# Autodesk Inventor assembly: 51200
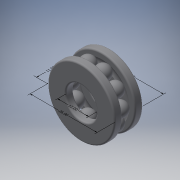
[picture p0: Inventor's stored thumbnail of the model, 180x180]
Saved by Autodesk Inventor 2019 (Build 230136000, 136)
## iProperties
Category: PARTsolutions
Company: NSK_RB
Created: 2023-01-10
Part Number: 51200
Catalog Web Link: www.cadenas.de
Description: With Flat Seet-
Vendor: NSK_RB
Document SubType Name: Assembly
Designer: psAdmin
Manufacturer: NSK_RB
Mass: 28 g
Surface Area: 32.9305 cm^2
Volume: 3.43224 cm^3
Density: 8.15795 g/cm^3
Title: 51200
Author: Cadenas PARTsolutions
PSOL_IDENT_0: {$CADENAS_DATA/23d-libs/nsk_rb/roller_bearings/thrust_bearings/single_direction_tbb/with_flat_seet_a
PSOL_IDENT_1: smtab.prj},174 {VTYP=3D},{STYP=ASSTAB},{NB=51200},{LINA=51200},{NN=With Flat Seet},{DATE=27.09.2022
PSOL_IDENT_2: 23:23:10},{GEOMDATE=23.08.2022 10:47:17},{VERSION=},{LINEID=6260},{WBVAR=},{WBNUMERIC=}  {NB=51200},
PSOL_IDENT_3: {LINA=51200},{KT=DUMMY},{IDNR=},{STAN=Standard},{NO=2},{ORDER=51200},{SD=10},{D=26},{T=11},{T3=11.6}
PSOL_IDENT_4: ,{T4=13},{SR=0.6},{CAN=12800},{COAN=17100},{CA=1300},{COA=1740},{GRE=6000},{OIL=9000},{SD1=26},{D1=1
PSOL_IDENT_5: 2},{D2=18},{D3=28},{SB=3.5},{A=8.5},{R=22},{SDA=20},{DA=16},{SRA=0.6},{MASS=0.028},{PPATH=with_flat_
PSOL_IDENT_6: seet_asmtpl.prj},{N=10},{DIST=1.233}
NB: 51200
NN: With Flat Seet
NBSYN: $ORDER.
LINA: 51200
CATALOG: NSK Rolling Bearing
ORDER: 51200
SD: 10
D: 26
T: 11
SR: 0.6
CAN: 12800
COAN: 17100
CA: 1300
COA: 1740
GRE: 6000
OIL: 9000
SD1: 26
D1: 12
SDA: 20
DA: 16
SRA: 0.6
MASS: 0.028
SUPPLIER: NSK_RB
ARTICLENO: 51200
BOMINFO: 51200
CREATOR: CADENAS GmbH
## Documents named in this file (4)
- e:\temp\worker_COMMON_5\temp\tmp_3544_152_Vz12m\format_0\51200.iam
- e:\temp\worker_COMMON_5\temp\tmp_3544_152_Vz12m\format_0\51200 Housing washer.ipt
- e:\temp\worker_COMMON_5\temp\tmp_3544_152_Vz12m\format_0\51200 Shaft washer.ipt
- e:\temp\worker_COMMON_5\temp\tmp_3544_152_Vz12m\format_0\51200 Ball.ipt
## Components (12 placed, 3 different names)
1. 51200 Housing washer:1 — HW_SW_XY@1 <-> SW_HW_XY@2, HW_SW_Z@1 <-> SW_HW_Z@2, HW_B_1_XY@1 <-> B_HW_XY@3, HW_B_1_Z@1 <-> B_HW_Z@3, HW_B_1_YZ@1 <-> B_HW_YZ@3, HW_B_2_XY@1 <-> B_HW_XY@4, HW_B_2_Z@1 <-> B_HW_Z@4, HW_B_2_YZ@1 <-> B_HW_YZ@4, HW_B_3_XY@1 <-> B_HW_XY@5, HW_B_3_Z@1 <-> B_HW_Z@5, HW_B_3_YZ@1 <-> B_HW_YZ@5, HW_B_4_XY@1 <-> B_HW_XY@6, HW_B_4_Z@1 <-> B_HW_Z@6, HW_B_4_YZ@1 <-> B_HW_YZ@6, HW_B_5_XY@1 <-> B_HW_XY@7, HW_B_5_Z@1 <-> B_HW_Z@7, HW_B_5_YZ@1 <-> B_HW_YZ@7, HW_B_6_XY@1 <-> B_HW_XY@8, HW_B_6_Z@1 <-> B_HW_Z@8, HW_B_6_YZ@1 <-> B_HW_YZ@8, HW_B_7_XY@1 <-> B_HW_XY@9, HW_B_7_Z@1 <-> B_HW_Z@9, HW_B_7_YZ@1 <-> B_HW_YZ@9, HW_B_8_XY@1 <-> B_HW_XY@10, HW_B_8_Z@1 <-> B_HW_Z@10, HW_B_8_YZ@1 <-> B_HW_YZ@10, HW_B_9_XY@1 <-> B_HW_XY@11, HW_B_9_Z@1 <-> B_HW_Z@11, HW_B_9_YZ@1 <-> B_HW_YZ@11, HW_B_10_XY@1 <-> B_HW_XY@12, HW_B_10_Z@1 <-> B_HW_Z@12, HW_B_10_YZ@1 <-> B_HW_YZ@12
2. 51200 Shaft washer:1 — HW_SW_XY@1 <-> SW_HW_XY@2, HW_SW_Z@1 <-> SW_HW_Z@2
3. 51200 Ball:1 — HW_B_1_XY@1 <-> B_HW_XY@3, HW_B_1_Z@1 <-> B_HW_Z@3, HW_B_1_YZ@1 <-> B_HW_YZ@3
4. 51200 Ball:2 — HW_B_2_XY@1 <-> B_HW_XY@4, HW_B_2_Z@1 <-> B_HW_Z@4, HW_B_2_YZ@1 <-> B_HW_YZ@4
5. 51200 Ball:3 — HW_B_3_XY@1 <-> B_HW_XY@5, HW_B_3_Z@1 <-> B_HW_Z@5, HW_B_3_YZ@1 <-> B_HW_YZ@5
6. 51200 Ball:4 — HW_B_4_XY@1 <-> B_HW_XY@6, HW_B_4_Z@1 <-> B_HW_Z@6, HW_B_4_YZ@1 <-> B_HW_YZ@6
7. 51200 Ball:5 — HW_B_5_XY@1 <-> B_HW_XY@7, HW_B_5_Z@1 <-> B_HW_Z@7, HW_B_5_YZ@1 <-> B_HW_YZ@7
8. 51200 Ball:6 — HW_B_6_XY@1 <-> B_HW_XY@8, HW_B_6_Z@1 <-> B_HW_Z@8, HW_B_6_YZ@1 <-> B_HW_YZ@8
9. 51200 Ball:7 — HW_B_7_XY@1 <-> B_HW_XY@9, HW_B_7_Z@1 <-> B_HW_Z@9, HW_B_7_YZ@1 <-> B_HW_YZ@9
10. 51200 Ball:8 — HW_B_8_XY@1 <-> B_HW_XY@10, HW_B_8_Z@1 <-> B_HW_Z@10, HW_B_8_YZ@1 <-> B_HW_YZ@10
11. 51200 Ball:9 — HW_B_9_XY@1 <-> B_HW_XY@11, HW_B_9_Z@1 <-> B_HW_Z@11, HW_B_9_YZ@1 <-> B_HW_YZ@11
12. 51200 Ball:10 — HW_B_10_XY@1 <-> B_HW_XY@12, HW_B_10_Z@1 <-> B_HW_Z@12, HW_B_10_YZ@1 <-> B_HW_YZ@12
## Relationships (32: Mate 21, Angle 10, Flush 1)
- HW_SW_XY@1 <-> SW_HW_XY@2 [Flush]: 51200 Housing washer:1 ↔ 51200 Shaft washer:1
- HW_SW_Z@1 <-> SW_HW_Z@2 [Mate]: 51200 Housing washer:1 ↔ 51200 Shaft washer:1
- HW_B_1_XY@1 <-> B_HW_XY@3 [Mate]: 51200 Housing washer:1 ↔ 51200 Ball:1
- HW_B_1_Z@1 <-> B_HW_Z@3 [Mate]: 51200 Housing washer:1 ↔ 51200 Ball:1
- HW_B_1_YZ@1 <-> B_HW_YZ@3 [Angle] (0 deg): 51200 Housing washer:1 ↔ 51200 Ball:1
- HW_B_2_XY@1 <-> B_HW_XY@4 [Mate]: 51200 Housing washer:1 ↔ 51200 Ball:2
- HW_B_2_Z@1 <-> B_HW_Z@4 [Mate]: 51200 Housing washer:1 ↔ 51200 Ball:2
- HW_B_2_YZ@1 <-> B_HW_YZ@4 [Angle] (0 deg): 51200 Housing washer:1 ↔ 51200 Ball:2
- HW_B_3_XY@1 <-> B_HW_XY@5 [Mate]: 51200 Housing washer:1 ↔ 51200 Ball:3
- HW_B_3_Z@1 <-> B_HW_Z@5 [Mate]: 51200 Housing washer:1 ↔ 51200 Ball:3
- HW_B_3_YZ@1 <-> B_HW_YZ@5 [Angle] (0 deg): 51200 Housing washer:1 ↔ 51200 Ball:3
- HW_B_4_XY@1 <-> B_HW_XY@6 [Mate]: 51200 Housing washer:1 ↔ 51200 Ball:4
- HW_B_4_Z@1 <-> B_HW_Z@6 [Mate]: 51200 Housing washer:1 ↔ 51200 Ball:4
- HW_B_4_YZ@1 <-> B_HW_YZ@6 [Angle] (0 deg): 51200 Housing washer:1 ↔ 51200 Ball:4
- HW_B_5_XY@1 <-> B_HW_XY@7 [Mate]: 51200 Housing washer:1 ↔ 51200 Ball:5
- HW_B_5_Z@1 <-> B_HW_Z@7 [Mate]: 51200 Housing washer:1 ↔ 51200 Ball:5
- HW_B_5_YZ@1 <-> B_HW_YZ@7 [Angle] (0 deg): 51200 Housing washer:1 ↔ 51200 Ball:5
- HW_B_6_XY@1 <-> B_HW_XY@8 [Mate]: 51200 Housing washer:1 ↔ 51200 Ball:6
- HW_B_6_Z@1 <-> B_HW_Z@8 [Mate]: 51200 Housing washer:1 ↔ 51200 Ball:6
- HW_B_6_YZ@1 <-> B_HW_YZ@8 [Angle] (0 deg): 51200 Housing washer:1 ↔ 51200 Ball:6
- HW_B_7_XY@1 <-> B_HW_XY@9 [Mate]: 51200 Housing washer:1 ↔ 51200 Ball:7
- HW_B_7_Z@1 <-> B_HW_Z@9 [Mate]: 51200 Housing washer:1 ↔ 51200 Ball:7
- HW_B_7_YZ@1 <-> B_HW_YZ@9 [Angle] (0 deg): 51200 Housing washer:1 ↔ 51200 Ball:7
- HW_B_8_XY@1 <-> B_HW_XY@10 [Mate]: 51200 Housing washer:1 ↔ 51200 Ball:8
- HW_B_8_Z@1 <-> B_HW_Z@10 [Mate]: 51200 Housing washer:1 ↔ 51200 Ball:8
- HW_B_8_YZ@1 <-> B_HW_YZ@10 [Angle] (0 deg): 51200 Housing washer:1 ↔ 51200 Ball:8
- HW_B_9_XY@1 <-> B_HW_XY@11 [Mate]: 51200 Housing washer:1 ↔ 51200 Ball:9
- HW_B_9_Z@1 <-> B_HW_Z@11 [Mate]: 51200 Housing washer:1 ↔ 51200 Ball:9
- HW_B_9_YZ@1 <-> B_HW_YZ@11 [Angle] (0 deg): 51200 Housing washer:1 ↔ 51200 Ball:9
- HW_B_10_XY@1 <-> B_HW_XY@12 [Mate]: 51200 Housing washer:1 ↔ 51200 Ball:10
- HW_B_10_Z@1 <-> B_HW_Z@12 [Mate]: 51200 Housing washer:1 ↔ 51200 Ball:10
- HW_B_10_YZ@1 <-> B_HW_YZ@12 [Angle] (0 deg): 51200 Housing washer:1 ↔ 51200 Ball:10
